# Autodesk Inventor assembly: Effector_Arm
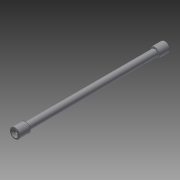
[picture p0: Inventor's stored thumbnail of the model, 180x180]
Saved by Autodesk Inventor 2014 (Build 180170000, 170)
## iProperties
Created: 2014-08-27
Part Number: Effector_Arm
Document SubType Name: Assembly
Designer: ThatOtherGuy
Author: ThatOtherGuy
## Documents named in this file (4)
- C:\Users\ThatOtherGuy\Documents\Inventor\KosselCNC1515\Effector\Effector_Arm.iam
- C:\Users\ThatOtherGuy\Documents\Inventor\KosselCNC1515\Joints\Joint_Magnet.ipt
- C:\Users\ThatOtherGuy\Documents\Inventor\KosselCNC1515\Effector\2219_Arrowshaft.ipt
- C:\Users\ThatOtherGuy\Documents\Inventor\KosselCNC1515\Effector\Arrow_Adapter.ipt
## Components (5 placed, 3 different names)
1. 2219_Arrowshaft:1 — Mate:1, Mate:3, Mate:4
2. Joint_Magnet:1 — Mate:1, Mate:2, Mate:3, Insert:5
3. Joint_Magnet:2 — Insert:4, Mate:2
4. Arrow_Adapter:1 — Insert:5
5. Arrow_Adapter:2 — Insert:4, Mate:4
## Relationships (6: Mate 4, Insert 2)
- Mate:1: 2219_Arrowshaft:1 ↔ Joint_Magnet:1
- Insert:4: Joint_Magnet:2 ↔ Arrow_Adapter:2
- Mate:2 (-185 mm): Joint_Magnet:1 ↔ Joint_Magnet:2
- Mate:3 (1.5 mm): 2219_Arrowshaft:1 ↔ Joint_Magnet:1
- Mate:4: 2219_Arrowshaft:1 ↔ Arrow_Adapter:2
- Insert:5: Joint_Magnet:1 ↔ Arrow_Adapter:1
